# Autodesk Inventor assembly: BoltWasher3x18
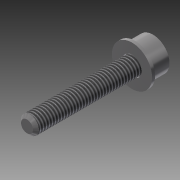
[picture p0: Inventor's stored thumbnail of the model, 180x180]
Saved by Autodesk Inventor 2016 (Build 200138000, 138)
## iProperties
Category: Hardware
Created: 2015-03-14
Part Number: BoltWasher3x18
Document SubType Name: Assembly
Designer: Jack
Mass: 1.60304 g
Surface Area: 3.53213 cm^2
Volume: 0.200244 cm^3
Density: 8.00544 g/cm^3
Vendor: McMaster Carr
Author: Jack
Title: Bolt Washer 3x18
## Documents named in this file (3)
- C:\Users\Jack\ownCloud\Projects\CrossBot\InventorModel\Hardware\BoltWashers\BoltWasher3\BoltWasher3x18.iam
- C:\Users\Jack\ownCloud\Projects\CrossBot\InventorModel\Hardware\Bolts\SHCS\SHCS3\SHCS3x18.ipt
- C:\Users\Jack\ownCloud\Projects\CrossBot\InventorModel\Hardware\Wahsers\M3Washer.ipt
## Components (2 placed, 2 different names)
1. SHCS3x18:1 — Mate:1, Mate:2
2. M3Washer:1 — Mate:1, Mate:2
## Relationships (2: Mate 2)
- Mate:1: SHCS3x18:1 ↔ M3Washer:1
- Mate:2: SHCS3x18:1 ↔ M3Washer:1
